# Autodesk Inventor assembly: ASY NVPH-400 shredder
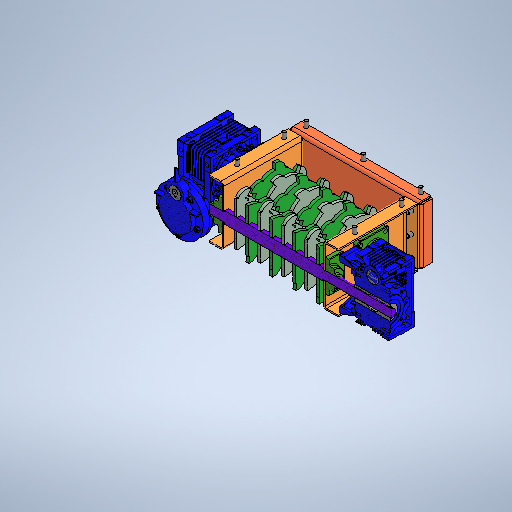
[picture p0: Inventor's stored thumbnail of the model, 512x512]
Saved by Autodesk Inventor 2025.1 (Build 291241020, 241B)
## iProperties
Created: 2024-12-13
Part Number: ASY NVPH-400 shredder
Document SubType Name: Assembly
Designer: user
Author: user
## Documents named in this file (7)
- C:\Users\user\YandexDisk-badmisterfox\домашниий пк\Inventor\NDM-VOS_powder_hopper\ASY NVPH-400 shredder.iam
- C:\Users\user\YandexDisk-badmisterfox\домашниий пк\Inventor\NDM-VOS_powder_hopper\ASY NVPH-200 shredder shaft full.iam
- C:\Users\user\YandexDisk-badmisterfox\домашниий пк\Inventor\NDM-VOS_powder_hopper\NDM-VOS 111 sredder wall .ipt
- C:\Users\user\YandexDisk-badmisterfox\домашниий пк\Inventor\NDM-VOS_powder_hopper\3d party\PCRV080-075SHFA_MS80B5\PCRV080-075SHFA_MS80B5\PCRV080-075SHFA_MS80B5.ipt
- C:\Users\user\YandexDisk-badmisterfox\домашниий пк\Inventor\NDM-VOS_powder_hopper\NDM-VOS 111 sredder wall _CPY.ipt
- C:\Users\user\YandexDisk-badmisterfox\домашниий пк\Inventor\Content Center Files\en-US\ISO 4017(1)\ISO 4017 - M12 x 25 - ISO.ipt
- C:\Users\user\YandexDisk-badmisterfox\домашниий пк\Inventor\NDM-VOS_powder_hopper\NDM-VOS dummy Disc Harrow Pillow block bearing mount Assembly.ipt
## Components (48 placed, 6 different names)
1. ASY NVPH-200 shredder shaft full:1 [sub-assembly] — Rotational:1
2. ASY NVPH-200 shredder shaft full:2 [sub-assembly] — Rotational:2
3. NDM-VOS 111 sredder wall :1 — Rigid:1, Rigid:3, Insert:13, Insert:14, Insert:15, Insert:16, Insert:17, Insert:18, Flush:1, Rigid:6, Rigid:7, Rotational:1, Rotational:3
4. NDM-VOS 111 sredder wall :2 — Rigid:2, Insert:19, Insert:20, Insert:21, Insert:22, Insert:23, Insert:24, Rigid:8, Rigid:9, Rigid:10, Rotational:2
5. PCRV080-075SHFA_MS80B5:1 — Rotational:3
6. PCRV080-075SHFA_MS80B5:2 — Rigid:10
7. NDM-VOS 112 sredder wall sub:1 — Rigid:1, Rigid:2, Insert:1, Insert:2, Insert:3, Insert:4, Insert:5, Insert:6, Insert:7, Insert:8, Insert:9, Insert:10, Insert:11, Insert:12, Mate:1, Mate:2
8. NDM-VOS 112 sredder wall sub:2 — Rigid:3, Insert:25, Insert:26, Insert:27, Insert:28, Insert:29, Insert:30, Insert:31, Insert:32, Insert:33, Insert:34, Insert:35, Insert:36
9. NDM-VOS dummy Disc Harrow Pillow block bearing mount Assembly:1 — Rigid:6
10. NDM-VOS dummy Disc Harrow Pillow block bearing mount Assembly:2 — Rigid:7
11. NDM-VOS dummy Disc Harrow Pillow block bearing mount Assembly:3 — Rigid:8
12. NDM-VOS dummy Disc Harrow Pillow block bearing mount Assembly:4 — Rigid:9
13. ISO 4017 M12 x 25:1 — Insert:1
14. ISO 4017 M12 x 25:2 — Insert:2
15. ISO 4017 M12 x 25:3 — Insert:3
16. ISO 4017 M12 x 25:4 — Insert:4
17. ISO 4017 M12 x 25:5 — Insert:5
18. ISO 4017 M12 x 25:6 — Insert:6
19. ISO 4017 M12 x 25:7 — Insert:7
20. ISO 4017 M12 x 25:8 — Insert:8
21. ISO 4017 M12 x 25:9 — Insert:9
22. ISO 4017 M12 x 25:10 — Insert:10
23. ISO 4017 M12 x 25:11 — Insert:11
24. ISO 4017 M12 x 25:12 — Insert:12
25. ISO 4017 M12 x 25:13 — Insert:13
26. ISO 4017 M12 x 25:14 — Insert:14
27. ISO 4017 M12 x 25:15 — Insert:15
28. ISO 4017 M12 x 25:16 — Insert:16
29. ISO 4017 M12 x 25:17 — Insert:17
30. ISO 4017 M12 x 25:18 — Insert:18
31. ISO 4017 M12 x 25:19 — Insert:19
32. ISO 4017 M12 x 25:20 — Insert:20
33. ISO 4017 M12 x 25:21 — Insert:21
34. ISO 4017 M12 x 25:22 — Insert:22
35. ISO 4017 M12 x 25:23 — Insert:23
36. ISO 4017 M12 x 25:24 — Insert:24
37. ISO 4017 M12 x 25:25 — Insert:25
38. ISO 4017 M12 x 25:26 — Insert:26
39. ISO 4017 M12 x 25:27 — Insert:27
40. ISO 4017 M12 x 25:28 — Insert:28
41. ISO 4017 M12 x 25:29 — Insert:29
42. ISO 4017 M12 x 25:30 — Insert:30
43. ISO 4017 M12 x 25:31 — Insert:31
44. ISO 4017 M12 x 25:32 — Insert:32
45. ISO 4017 M12 x 25:33 — Insert:33
46. ISO 4017 M12 x 25:34 — Insert:34
47. ISO 4017 M12 x 25:35 — Insert:35
48. ISO 4017 M12 x 25:36 — Insert:36
## Relationships (50: Insert 36, WeldJoint 8, RevoluteJoint 3, Mate 2, Flush 1)
- Rigid:1 [WeldJoint]: NDM-VOS 111 sredder wall :1 ↔ NDM-VOS 112 sredder wall sub:1
- Rigid:2 [WeldJoint]: NDM-VOS 111 sredder wall :2 ↔ NDM-VOS 112 sredder wall sub:1
- Rigid:3 [WeldJoint]: NDM-VOS 111 sredder wall :1 ↔ NDM-VOS 112 sredder wall sub:2
- Insert:1: NDM-VOS 112 sredder wall sub:1 ↔ ISO 4017 M12 x 25:1
- Insert:2: NDM-VOS 112 sredder wall sub:1 ↔ ISO 4017 M12 x 25:2
- Insert:3: NDM-VOS 112 sredder wall sub:1 ↔ ISO 4017 M12 x 25:3
- Insert:4: NDM-VOS 112 sredder wall sub:1 ↔ ISO 4017 M12 x 25:4
- Insert:5: NDM-VOS 112 sredder wall sub:1 ↔ ISO 4017 M12 x 25:5
- Insert:6: NDM-VOS 112 sredder wall sub:1 ↔ ISO 4017 M12 x 25:6
- Insert:7: NDM-VOS 112 sredder wall sub:1 ↔ ISO 4017 M12 x 25:7
- Insert:8: NDM-VOS 112 sredder wall sub:1 ↔ ISO 4017 M12 x 25:8
- Insert:9: NDM-VOS 112 sredder wall sub:1 ↔ ISO 4017 M12 x 25:9
- Insert:10: NDM-VOS 112 sredder wall sub:1 ↔ ISO 4017 M12 x 25:10
- Insert:11: NDM-VOS 112 sredder wall sub:1 ↔ ISO 4017 M12 x 25:11
- Insert:12: NDM-VOS 112 sredder wall sub:1 ↔ ISO 4017 M12 x 25:12
- Insert:13: NDM-VOS 111 sredder wall :1 ↔ ISO 4017 M12 x 25:13
- Insert:14: NDM-VOS 111 sredder wall :1 ↔ ISO 4017 M12 x 25:14
- Insert:15: NDM-VOS 111 sredder wall :1 ↔ ISO 4017 M12 x 25:15
- Insert:16: NDM-VOS 111 sredder wall :1 ↔ ISO 4017 M12 x 25:16
- Insert:17: NDM-VOS 111 sredder wall :1 ↔ ISO 4017 M12 x 25:17
- Insert:18: NDM-VOS 111 sredder wall :1 ↔ ISO 4017 M12 x 25:18
- Insert:19: NDM-VOS 111 sredder wall :2 ↔ ISO 4017 M12 x 25:19
- Insert:20: NDM-VOS 111 sredder wall :2 ↔ ISO 4017 M12 x 25:20
- Insert:21: NDM-VOS 111 sredder wall :2 ↔ ISO 4017 M12 x 25:21
- Insert:22: NDM-VOS 111 sredder wall :2 ↔ ISO 4017 M12 x 25:22
- Insert:23: NDM-VOS 111 sredder wall :2 ↔ ISO 4017 M12 x 25:23
- Insert:24: NDM-VOS 111 sredder wall :2 ↔ ISO 4017 M12 x 25:24
- Insert:25: NDM-VOS 112 sredder wall sub:2 ↔ ISO 4017 M12 x 25:25
- Insert:26: NDM-VOS 112 sredder wall sub:2 ↔ ISO 4017 M12 x 25:26
- Insert:27: NDM-VOS 112 sredder wall sub:2 ↔ ISO 4017 M12 x 25:27
- Insert:28: NDM-VOS 112 sredder wall sub:2 ↔ ISO 4017 M12 x 25:28
- Insert:29: NDM-VOS 112 sredder wall sub:2 ↔ ISO 4017 M12 x 25:29
- Insert:30: NDM-VOS 112 sredder wall sub:2 ↔ ISO 4017 M12 x 25:30
- Insert:31: NDM-VOS 112 sredder wall sub:2 ↔ ISO 4017 M12 x 25:31
- Insert:32: NDM-VOS 112 sredder wall sub:2 ↔ ISO 4017 M12 x 25:32
- Insert:33: NDM-VOS 112 sredder wall sub:2 ↔ ISO 4017 M12 x 25:33
- Insert:34: NDM-VOS 112 sredder wall sub:2 ↔ ISO 4017 M12 x 25:34
- Insert:35: NDM-VOS 112 sredder wall sub:2 ↔ ISO 4017 M12 x 25:35
- Insert:36: NDM-VOS 112 sredder wall sub:2 ↔ ISO 4017 M12 x 25:36
- Mate:1: NDM-VOS 112 sredder wall sub:1
- Mate:2: NDM-VOS 112 sredder wall sub:1
- Flush:1: NDM-VOS 111 sredder wall :1
- Rigid:6 [WeldJoint]: NDM-VOS 111 sredder wall :1 ↔ NDM-VOS dummy Disc Harrow Pillow block bearing mount Assembly:1
- Rigid:7 [WeldJoint]: NDM-VOS 111 sredder wall :1 ↔ NDM-VOS dummy Disc Harrow Pillow block bearing mount Assembly:2
- Rigid:8 [WeldJoint]: NDM-VOS 111 sredder wall :2 ↔ NDM-VOS dummy Disc Harrow Pillow block bearing mount Assembly:3
- Rigid:9 [WeldJoint]: NDM-VOS 111 sredder wall :2 ↔ NDM-VOS dummy Disc Harrow Pillow block bearing mount Assembly:4
- Rigid:10 [WeldJoint] (50 mm): NDM-VOS 111 sredder wall :2 ↔ PCRV080-075SHFA_MS80B5:2
- Rotational:1 [RevoluteJoint] (-3 mm): ASY NVPH-200 shredder shaft full:1 ↔ NDM-VOS 111 sredder wall :1
- Rotational:2 [RevoluteJoint] (-3 mm): ASY NVPH-200 shredder shaft full:2 ↔ NDM-VOS 111 sredder wall :2
- Rotational:3 [RevoluteJoint] (50 mm): NDM-VOS 111 sredder wall :1 ↔ PCRV080-075SHFA_MS80B5:1
